# Autodesk Inventor assembly: IRB 4600-40_2.55
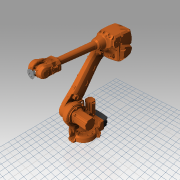
[picture p0: Inventor's stored thumbnail of the model, 180x180]
Saved by Autodesk Inventor 2017 (Build 210142000, 142)
## iProperties
Created: 2017-02-16
Part Number: IRB 4600-40_2.55
Document SubType Name: Assembly
Designer: User
Mass: 173320 g
Surface Area: 52582.7 cm^2
Volume: 173320 cm^3
Density: 1 g/cm^3
Author: User
## Documents named in this file (9)
- C:\Projetos Mecânicos\ABB\ABB4600\IRB 4600-40_2.55.iam
- C:\Projetos Mecânicos\ABB\ABB4600\IRB 4600-40_2.55.ipt
- C:\Projetos Mecânicos\ABB\ABB4600\IRB 4600-40_2.55_1.ipt
- C:\Projetos Mecânicos\ABB\ABB4600\IRB 4600-40_2.55_2.ipt
- C:\Projetos Mecânicos\ABB\ABB4600\IRB 4600-40_2.55_3.ipt
- C:\Projetos Mecânicos\ABB\ABB4600\IRB 4600-40_2.55_4.ipt
- C:\Projetos Mecânicos\ABB\ABB4600\IRB 4600-40_2.55_5.ipt
- C:\Projetos Mecânicos\ABB\ABB4600\IRB 4600-40_2.55_6.ipt
- C:\Projetos Mecânicos\ABB\ABB4600\IRB 4600-40_2.55_7.ipt
## Components (8 placed, 8 different names)
1. IRB 4600-40_2.55:1 — Mate:11, Mate:13
2. IRB 4600-40_2.55_1:1 — Mate:9, Mate:10, Mate:11, Mate:12, Mate:13
3. IRB 4600-40_2.55_2:1 — Mate:7, Mate:8, Mate:9, Mate:10, Mate:12, Angle:2
4. IRB 4600-40_2.55_3:1 — Mate:5, Mate:6, Mate:7, Mate:8
5. IRB 4600-40_2.55_4:1 — Mate:3, Mate:4, Mate:5, Mate:6
6. IRB 4600-40_2.55_5:1 — Mate:1, Mate:2, Mate:3, Mate:4, Angle:1
7. IRB 4600-40_2.55_6:1 — Mate:1, Mate:2, Angle:1, Mate:14, Mate:15, Mate:16, Mate:17
8. IRB 4600-40_2.55_7:1 — Mate:15, Mate:16, Mate:17
## Relationships (19: Mate 17, Angle 2)
- Mate:1: IRB 4600-40_2.55_5:1 ↔ IRB 4600-40_2.55_6:1
- Mate:2: IRB 4600-40_2.55_5:1 ↔ IRB 4600-40_2.55_6:1
- Mate:3: IRB 4600-40_2.55_4:1 ↔ IRB 4600-40_2.55_5:1
- Mate:4 (1.5 mm): IRB 4600-40_2.55_4:1 ↔ IRB 4600-40_2.55_5:1
- Mate:5: IRB 4600-40_2.55_3:1 ↔ IRB 4600-40_2.55_4:1
- Mate:6: IRB 4600-40_2.55_3:1 ↔ IRB 4600-40_2.55_4:1
- Mate:7: IRB 4600-40_2.55_2:1 ↔ IRB 4600-40_2.55_3:1
- Mate:8: IRB 4600-40_2.55_2:1 ↔ IRB 4600-40_2.55_3:1
- Mate:9: IRB 4600-40_2.55_1:1 ↔ IRB 4600-40_2.55_2:1
- Mate:10: IRB 4600-40_2.55_1:1 ↔ IRB 4600-40_2.55_2:1
- Mate:11: IRB 4600-40_2.55:1 ↔ IRB 4600-40_2.55_1:1
- Mate:12: IRB 4600-40_2.55_1:1 ↔ IRB 4600-40_2.55_2:1
- Mate:13: IRB 4600-40_2.55:1 ↔ IRB 4600-40_2.55_1:1
- Angle:1 (0 deg): IRB 4600-40_2.55_5:1 ↔ IRB 4600-40_2.55_6:1
- Angle:2 (-90 deg): IRB 4600-40_2.55_2:1
- Mate:14: IRB 4600-40_2.55_6:1
- Mate:15: IRB 4600-40_2.55_6:1 ↔ IRB 4600-40_2.55_7:1
- Mate:16: IRB 4600-40_2.55_6:1 ↔ IRB 4600-40_2.55_7:1
- Mate:17: IRB 4600-40_2.55_6:1 ↔ IRB 4600-40_2.55_7:1
